# Autodesk Inventor assembly: Elevator
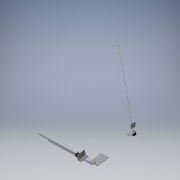
[picture p0: Inventor's stored thumbnail of the model, 180x180]
Saved by Autodesk Inventor 2017 (Build 210142000, 142)
## iProperties
Created: 2016-12-12
Part Number: Elevator
Document SubType Name: Assembly
Designer: umr
Mass: 4376.08 g
Surface Area: 10170.9 cm^2
Volume: 1553.17 cm^3
Density: 2.81752 g/cm^3
Author: umr
## Documents named in this file (13)
- D:\SeniorProject\Models2\Gantry\GantryDown.iam
- D:\SeniorProject\Models2\Gantry\M5 Screw with Tee Nut.iam
- D:\SeniorProject\Models2\Gantry\L_Fixer.ipt
- D:\SeniorProject\Models2\Gantry\ScrewDriver.ipt
- D:\SeniorProject\Models2\Gantry\Motor.ipt
- D:\SeniorProject\Models2\Gantry\Motor Mount Plate.ipt
- D:\SeniorProject\Models2\Gantry\Driveshaft.ipt
- D:\SeniorProject\Models2\Gantry\5mm x 5mm Flexible Coupling.ipt
- D:\SeniorProject\Models2\Gantry\GT2 20 Tooth Pulley.ipt
- D:\SeniorProject\Models2\MotorPlate.ipt
- D:\SeniorProject\Models2\Gantry\GantryPlate_v3.ipt
- D:\SeniorProject\Models2\30x60Sigma.ipt
- D:\SeniorProject\Models2\WheelAssembly\OurWheelAssembly.iam
## Components (24 placed, 12 different names)
1. L_Fixer:1 — Mate:152, Mate:153, Mate:154, Mate:155, Flush:1, Flush:2
2. ScrewDriver:1 — Mate:72, Mate:73
3. Motor:1 — Mate:72, Mate:73, Mate:155, Flush:1, Flush:2
4. Motor Mount Plate:1 — Mate:88, Mate:89, Mate:90, Mate:91
5. M5 Screw with Tee Nut:15 [sub-assembly] — Mate:89, Mate:91
6. M5 Screw with Tee Nut:16 [sub-assembly] — Mate:90
7. M5 Screw with Tee Nut:17 [sub-assembly] — Mate:88
8. Motor:2 — Mate:140, Mate:141, Mate:145
9. 5mm x 5mm Flexible Coupling:1 — Mate:97
10. Driveshaft:1 — Mate:97, Mate:145, Mate:146, Mate:147
11. GT2 20 Tooth Pulley:1 — Mate:147
12. M5 Screw with Tee Nut:18 [sub-assembly] — Mate:143
13. M5 Screw with Tee Nut:19 [sub-assembly] — Mate:142
14. M5 Screw with Tee Nut:20 [sub-assembly] — Mate:144
15. MotorPlate:1 — Mate:140, Mate:141, Mate:142, Mate:143, Mate:144, Mate:146
16. GantryPlate_v3:1 — Mate:167, Mate:168, Mate:172, Mate:173, Mate:174, Mate:175, Mate:176
17. 30x60Sigma:1 — Mate:148, Mate:149, Mate:150, Mate:151, Mate:154, Mate:157, Mate:158, Mate:159, Mate:160, Mate:165, Mate:166, Mate:170, Mate:171, Mate:174
18. M5 Screw with Tee Nut:21 [sub-assembly] — Mate:148, Mate:149, Mate:152
19. M5 Screw with Tee Nut:22 [sub-assembly] — Mate:150, Mate:151, Mate:153
20. M5 Screw with Tee Nut:24 [sub-assembly] — Mate:157, Mate:171, Mate:173
21. M5 Screw with Tee Nut:25 [sub-assembly] — Mate:158, Mate:170, Mate:172
22. M5 Screw with Tee Nut:26 [sub-assembly] — Mate:159, Mate:165, Mate:167
23. M5 Screw with Tee Nut:27 [sub-assembly] — Mate:160, Mate:166, Mate:168
24. OurWheelAssembly:1 [sub-assembly] — Mate:175, Mate:176
## Relationships (40: Mate 38, Flush 2)
- Mate:72: ScrewDriver:1 ↔ Motor:1
- Mate:73: ScrewDriver:1 ↔ Motor:1
- Mate:88: Motor Mount Plate:1 ↔ M5 Screw with Tee Nut:17
- Mate:89: Motor Mount Plate:1 ↔ M5 Screw with Tee Nut:15
- Mate:90: Motor Mount Plate:1 ↔ M5 Screw with Tee Nut:16
- Mate:91: Motor Mount Plate:1 ↔ M5 Screw with Tee Nut:15
- Mate:97: 5mm x 5mm Flexible Coupling:1 ↔ Driveshaft:1
- Mate:140: Motor:2 ↔ MotorPlate:1
- Mate:141: Motor:2 ↔ MotorPlate:1
- Mate:142: M5 Screw with Tee Nut:19 ↔ MotorPlate:1
- Mate:143: M5 Screw with Tee Nut:18 ↔ MotorPlate:1
- Mate:144: M5 Screw with Tee Nut:20 ↔ MotorPlate:1
- Mate:145: Motor:2 ↔ Driveshaft:1
- Mate:146: Driveshaft:1 ↔ MotorPlate:1
- Mate:147: Driveshaft:1 ↔ GT2 20 Tooth Pulley:1
- Mate:148: 30x60Sigma:1 ↔ M5 Screw with Tee Nut:21
- Mate:149: 30x60Sigma:1 ↔ M5 Screw with Tee Nut:21
- Mate:150: 30x60Sigma:1 ↔ M5 Screw with Tee Nut:22
- Mate:151: 30x60Sigma:1 ↔ M5 Screw with Tee Nut:22
- Mate:152: L_Fixer:1 ↔ M5 Screw with Tee Nut:21
- Mate:153: L_Fixer:1 ↔ M5 Screw with Tee Nut:22
- Mate:154: L_Fixer:1 ↔ 30x60Sigma:1
- Mate:155: L_Fixer:1 ↔ Motor:1
- Flush:1 (-10 mm): L_Fixer:1 ↔ Motor:1
- Flush:2 (10 mm): L_Fixer:1 ↔ Motor:1
- Mate:157: 30x60Sigma:1 ↔ M5 Screw with Tee Nut:24
- Mate:158: 30x60Sigma:1 ↔ M5 Screw with Tee Nut:25
- Mate:159: 30x60Sigma:1 ↔ M5 Screw with Tee Nut:26
- Mate:160: 30x60Sigma:1 ↔ M5 Screw with Tee Nut:27
- Mate:165 (3 mm): 30x60Sigma:1 ↔ M5 Screw with Tee Nut:26
- Mate:166 (3 mm): 30x60Sigma:1 ↔ M5 Screw with Tee Nut:27
- Mate:167: GantryPlate_v3:1 ↔ M5 Screw with Tee Nut:26
- Mate:168: GantryPlate_v3:1 ↔ M5 Screw with Tee Nut:27
- Mate:170 (3 mm): 30x60Sigma:1 ↔ M5 Screw with Tee Nut:25
- Mate:171 (3 mm): 30x60Sigma:1 ↔ M5 Screw with Tee Nut:24
- Mate:172: GantryPlate_v3:1 ↔ M5 Screw with Tee Nut:25
- Mate:173: GantryPlate_v3:1 ↔ M5 Screw with Tee Nut:24
- Mate:174: GantryPlate_v3:1 ↔ 30x60Sigma:1
- Mate:175: GantryPlate_v3:1 ↔ OurWheelAssembly:1
- Mate:176: GantryPlate_v3:1 ↔ OurWheelAssembly:1
